# Autodesk Inventor assembly: FlatSat Assembly
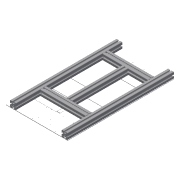
[picture p0: Inventor's stored thumbnail of the model, 180x180]
Saved by Autodesk Inventor 2018 (Build 220112000, 112)
## iProperties
Created: 2016-11-08
Part Number: FlatSat Assembly
Document SubType Name: Assembly
Designer: Jonis
Author: Jonis
## Documents named in this file (15)
- H:\CAD\FlatSat Release\FlatSat Assembly.iam
- H:\CAD\FlatSat Release\Profiles\item_0002603_Profil_8_40x40_L=370_1.ipt
- H:\CAD\FlatSat Release\Profiles\item_0002603_Profil_8_40x40_L=300_1.ipt
- H:\CAD\FlatSat Release\Profiles\item_0002603_Profil_8_40x40_L=700_2.ipt
- H:\CAD\FlatSat Release\Board\Base2.ipt
- H:\CAD\FlatSat Release\Board\Backbone2.ipt
- H:\CAD\FlatSat Release\Board\Spacing Layer 3.ipt
- H:\CAD\FlatSat Release\Subsystem Sheets\SupportsheetStandard2.ipt
- H:\CAD\FlatSat Release\Subsystem Sheets\SupportsheetCDH2.ipt
- H:\CAD\FlatSat Release\Subsystem Sheets\SupportsheetADCS2.ipt
- H:\CAD\FlatSat Release\Subsystem Sheets\SupportsheetEPS.ipt
- H:\CAD\FlatSat Release\Subsystem Sheets\SupportsheetMonitor.ipt
- H:\CAD\FlatSat Release\Board\FlatSat PCB 1\FlatSat Half1.iam
- H:\CAD\FlatSat Release\Board\FlatSat PCB 2\FlatSat Half 2.iam
- H:\CAD\FlatSat Release\Board\Spacing Layer 4.ipt
## Components (19 placed, 14 different names)
1. item_0002603_Profil_8_40x40_L=370_1:1 — Mate:1, Flush:1, Flush:2, Mate:2, Flush:3, Mate:5, Flush:9
2. item_0002603_Profil_8_40x40_L=300_1:1 — Mate:2, Flush:3, Flush:4, Flush:7, Flush:10
3. item_0002603_Profil_8_40x40_L=300_1:2 — Mate:1, Flush:1, Flush:2, Flush:4, Mate:3, Mate:4, Flush:5, Flush:6
4. item_0002603_Profil_8_40x40_L=700_2:1 — Mate:4, Flush:6, Flush:7, Flush:8, Mate:17, Flush:33, Mate:18, Flush:35, Flush:41, Mate:28, Flush:43, Flush:44, Mate:29, Flush:61
5. item_0002603_Profil_8_40x40_L=700_2:2 — Mate:3, Flush:5, Flush:8, Mate:20, Mate:21, Flush:36, Flush:37, Mate:22, Flush:39, Mate:27, Flush:42
6. Base2:1 — Mate:5, Flush:9, Flush:10, Mate:6, Flush:11, Flush:12
7. Backbone2:1 — Mate:6, Flush:11, Flush:12, Mate:7, Flush:13, Flush:14, Flush:75, Flush:76, Flush:77, Flush:78, Flush:79, Flush:80, Flush:81
8. Spacing Layer 3:1 — Mate:7, Flush:13, Flush:14, Mate:49, Mate:50, Flush:79
9. SupportsheetStandard2:1 — Mate:17, Flush:33, Mate:19
10. SupportsheetStandard2:2 — Mate:18, Flush:35, Mate:19, Mate:30
11. SupportsheetStandard2:3 — Mate:20, Flush:36, Mate:23
12. SupportsheetStandard2:4 — Mate:21, Flush:37, Mate:24
13. SupportsheetCDH2:1 — Mate:22, Flush:39, Mate:23, Mate:24
14. SupportsheetADCS2:1 — Mate:29, Mate:30, Flush:61
15. SupportsheetEPS:1 — Mate:27, Flush:41, Flush:42
16. SupportsheetMonitor:1 — Mate:28, Flush:43, Flush:44
17. FlatSat Half1:1 [sub-assembly] — Mate:49, Flush:75, Flush:76
18. FlatSat Half 2:1 [sub-assembly] — Mate:50, Flush:77, Flush:78
19. Spacing Layer 4:1 — Flush:80, Flush:81
## Relationships (52: Flush 31, Mate 21)
- Mate:1: item_0002603_Profil_8_40x40_L=370_1:1 ↔ item_0002603_Profil_8_40x40_L=300_1:2
- Flush:1: item_0002603_Profil_8_40x40_L=370_1:1 ↔ item_0002603_Profil_8_40x40_L=300_1:2
- Flush:2 (130 mm): item_0002603_Profil_8_40x40_L=370_1:1 ↔ item_0002603_Profil_8_40x40_L=300_1:2
- Mate:2: item_0002603_Profil_8_40x40_L=370_1:1 ↔ item_0002603_Profil_8_40x40_L=300_1:1
- Flush:3: item_0002603_Profil_8_40x40_L=370_1:1 ↔ item_0002603_Profil_8_40x40_L=300_1:1
- Flush:4: item_0002603_Profil_8_40x40_L=300_1:1 ↔ item_0002603_Profil_8_40x40_L=300_1:2
- Mate:3: item_0002603_Profil_8_40x40_L=300_1:2 ↔ item_0002603_Profil_8_40x40_L=700_2:2
- Mate:4: item_0002603_Profil_8_40x40_L=300_1:2 ↔ item_0002603_Profil_8_40x40_L=700_2:1
- Flush:5: item_0002603_Profil_8_40x40_L=300_1:2 ↔ item_0002603_Profil_8_40x40_L=700_2:2
- Flush:6: item_0002603_Profil_8_40x40_L=300_1:2 ↔ item_0002603_Profil_8_40x40_L=700_2:1
- Flush:7 (90 mm): item_0002603_Profil_8_40x40_L=300_1:1 ↔ item_0002603_Profil_8_40x40_L=700_2:1
- Flush:8: item_0002603_Profil_8_40x40_L=700_2:1 ↔ item_0002603_Profil_8_40x40_L=700_2:2
- Mate:5: item_0002603_Profil_8_40x40_L=370_1:1 ↔ Base2:1
- Flush:9 (-10 mm): item_0002603_Profil_8_40x40_L=370_1:1 ↔ Base2:1
- Flush:10 (28 mm): item_0002603_Profil_8_40x40_L=300_1:1 ↔ Base2:1
- Mate:6: Base2:1 ↔ Backbone2:1
- Flush:11 (26 mm): Base2:1 ↔ Backbone2:1
- Flush:12 (40 mm): Base2:1 ↔ Backbone2:1
- Mate:7: Backbone2:1 ↔ Spacing Layer 3:1
- Flush:13: Backbone2:1 ↔ Spacing Layer 3:1
- Flush:14: Backbone2:1 ↔ Spacing Layer 3:1
- Mate:17: item_0002603_Profil_8_40x40_L=700_2:1 ↔ SupportsheetStandard2:1
- Flush:33: item_0002603_Profil_8_40x40_L=700_2:1 ↔ SupportsheetStandard2:1
- Mate:18: item_0002603_Profil_8_40x40_L=700_2:1 ↔ SupportsheetStandard2:2
- Flush:35: item_0002603_Profil_8_40x40_L=700_2:1 ↔ SupportsheetStandard2:2
- Mate:19 (2 mm): SupportsheetStandard2:1 ↔ SupportsheetStandard2:2
- Mate:20: item_0002603_Profil_8_40x40_L=700_2:2 ↔ SupportsheetStandard2:3
- Mate:21: item_0002603_Profil_8_40x40_L=700_2:2 ↔ SupportsheetStandard2:4
- Flush:36: item_0002603_Profil_8_40x40_L=700_2:2 ↔ SupportsheetStandard2:3
- Flush:37: item_0002603_Profil_8_40x40_L=700_2:2 ↔ SupportsheetStandard2:4
- Mate:22: item_0002603_Profil_8_40x40_L=700_2:2 ↔ SupportsheetCDH2:1
- Flush:39: item_0002603_Profil_8_40x40_L=700_2:2 ↔ SupportsheetCDH2:1
- Mate:23 (2 mm): SupportsheetStandard2:3 ↔ SupportsheetCDH2:1
- Mate:24 (2 mm): SupportsheetStandard2:4 ↔ SupportsheetCDH2:1
- Mate:27: item_0002603_Profil_8_40x40_L=700_2:2 ↔ SupportsheetEPS:1
- Flush:41: item_0002603_Profil_8_40x40_L=700_2:1 ↔ SupportsheetEPS:1
- Flush:42: item_0002603_Profil_8_40x40_L=700_2:2 ↔ SupportsheetEPS:1
- Mate:28: item_0002603_Profil_8_40x40_L=700_2:1 ↔ SupportsheetMonitor:1
- Flush:43: item_0002603_Profil_8_40x40_L=700_2:1 ↔ SupportsheetMonitor:1
- Flush:44: item_0002603_Profil_8_40x40_L=700_2:1 ↔ SupportsheetMonitor:1
- Mate:29: item_0002603_Profil_8_40x40_L=700_2:1 ↔ SupportsheetADCS2:1
- Mate:30 (2 mm): SupportsheetStandard2:2 ↔ SupportsheetADCS2:1
- Flush:61 (26 mm): item_0002603_Profil_8_40x40_L=700_2:1 ↔ SupportsheetADCS2:1
- Mate:49: Spacing Layer 3:1 ↔ FlatSat Half1:1
- Flush:75: Backbone2:1 ↔ FlatSat Half1:1
- Flush:76: Backbone2:1 ↔ FlatSat Half1:1
- Mate:50: Spacing Layer 3:1 ↔ FlatSat Half 2:1
- Flush:77: Backbone2:1 ↔ FlatSat Half 2:1
- Flush:78: Backbone2:1 ↔ FlatSat Half 2:1
- Flush:79: Backbone2:1 ↔ Spacing Layer 3:1
- Flush:80: Backbone2:1 ↔ Spacing Layer 4:1
- Flush:81: Backbone2:1 ↔ Spacing Layer 4:1
